# Autodesk Inventor assembly: bushing_assembly
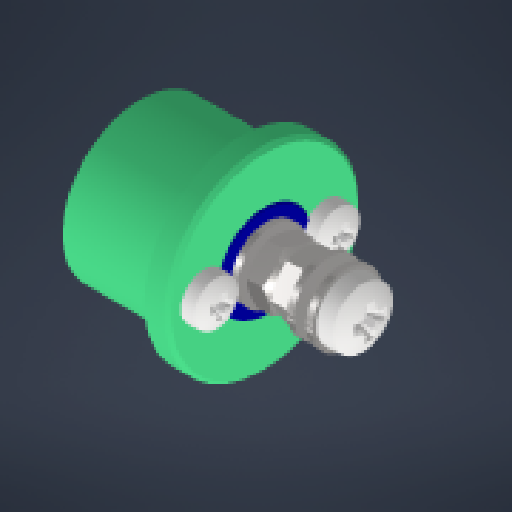
[picture p0: Inventor's stored thumbnail of the model, 512x512]
Saved by Autodesk Inventor 2024 (Build 280153000, 153)
## iProperties
Created: 2023-04-20
Part Number: bushing_assembly
Document SubType Name: Assembly
Designer: user
Author: user
## Documents named in this file (7)
- D:\Docs\Robot\3d\motor_assembly\bushing_assembly\bushing_assembly.iam
- D:\Docs\Robot\3d\motor_assembly\bushing_assembly\bushing.ipt
- D:\Docs\Robot\3d\motor_assembly\bushing_assembly\604zz_bearing.ipt
- C:\Users\user\Documents\Inventor\Content Center Files\R2024\ru-RU\DIN 125-1  A\DIN 125 - A 4,3.ipt
- C:\Users\user\Documents\Inventor\Content Center Files\R2024\ru-RU\DIN 7985 (H)\DIN 7985 (H) - M3x5-H.ipt
- C:\Users\user\Documents\Inventor\Content Center Files\R2024\ru-RU\DIN 934\DIN 934 - M4 x 0,7.ipt
- C:\Users\user\Documents\Inventor\Content Center Files\R2024\ru-RU\DIN 7985 (H)\DIN 7985 (H) - M4x16-H.ipt
## Components (10 placed, 6 different names)
1. bushing:1 — Совмещение:1, Совмещение:2, Совмещение:3, Вставка:1, Заподлицо:1, Вставка:2, Вставка:3
2. 604zz_bearing:1 — Вставка:1, Заподлицо:1, Вставка:7
3. DIN 7985 (H) M3x5-H:1 — Вставка:2
4. DIN 7985 (H) M3x5-H:2 — Вставка:3
5. DIN 934 - заменено на DIN EN 24032/28673/28674 M4:1 — Вставка:5, Вставка:8
6. DIN 934 - заменено на DIN EN 24032/28673/28674 M4:2 — Вставка:5, Вставка:6
7. DIN 125-1 A A 4,3:1 — Вставка:6, Вставка:10
8. DIN 125-1 A A 4,3:2 — Вставка:7, Вставка:8
9. DIN 7985 (H) M4x16-H:1 — Вставка:9
10. DIN 125-1 A A 4,3:3 — Вставка:9, Вставка:10
## Relationships (13: Insert 9, Mate 3, Flush 1)
- Совмещение:1 [Mate]: bushing:1
- Совмещение:2 [Mate]: bushing:1
- Совмещение:3 [Mate]: bushing:1
- Вставка:1 [Insert]: bushing:1 ↔ 604zz_bearing:1
- Заподлицо:1 [Flush]: bushing:1 ↔ 604zz_bearing:1
- Вставка:2 [Insert]: bushing:1 ↔ DIN 7985 (H) M3x5-H:1
- Вставка:3 [Insert]: bushing:1 ↔ DIN 7985 (H) M3x5-H:2
- Вставка:5 [Insert]: DIN 934 - заменено на DIN EN 24032/28673/28674 M4:1 ↔ DIN 934 - заменено на DIN EN 24032/28673/28674 M4:2
- Вставка:6 [Insert]: DIN 934 - заменено на DIN EN 24032/28673/28674 M4:2 ↔ DIN 125-1 A A 4,3:1
- Вставка:7 [Insert]: 604zz_bearing:1 ↔ DIN 125-1 A A 4,3:2
- Вставка:8 [Insert]: DIN 934 - заменено на DIN EN 24032/28673/28674 M4:1 ↔ DIN 125-1 A A 4,3:2
- Вставка:9 [Insert]: DIN 7985 (H) M4x16-H:1 ↔ DIN 125-1 A A 4,3:3
- Вставка:10 [Insert] (1.6 mm): DIN 125-1 A A 4,3:1 ↔ DIN 125-1 A A 4,3:3
